# Autodesk Inventor assembly: YZ-Axis Connection
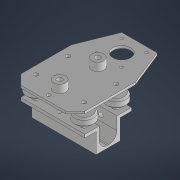
[picture p0: Inventor's stored thumbnail of the model, 180x180]
Saved by Autodesk Inventor 2022 (Build 260153000, 153)
## iProperties
Created: 2023-06-15
Part Number: YZ-Axis Connection
Document SubType Name: Assembly
Designer: Ryan Mitcham
Author: Ryan Mitcham
## Documents named in this file (5)
- C:\Users\Gaming\OneDrive\Documents\Inventor\XYZ-Gantry\YZ-Axis Connection\YZ-Axis Connection.iam
- C:\Users\Gaming\OneDrive\Documents\Inventor\XYZ-Gantry\YZ-Axis Connection\Back Plate.ipt
- C:\Users\Gaming\OneDrive\Documents\Inventor\XYZ-Gantry\YZ-Axis Connection\Back Plate Spacer.ipt
- C:\Users\Gaming\OneDrive\Documents\Inventor\XYZ-Gantry\YZ-Axis Connection\Wheel Mount.ipt
- C:\Users\Gaming\OneDrive\Documents\Inventor\XYZ-Gantry\Standard Parts\20x20 Extrusion Compatible Wheel - Dual Spacers.ipt
## Components (8 placed, 4 different names)
1. Back Plate:1 — Mate:1, Mate:2, Mate:3, Mate:4, Mate:5, Mate:6, Mate:7, Mate:8, Mate:9, Mate:10, Mate:11, Mate:12
2. Back Plate Spacer:1 — Mate:1, Mate:4
3. Back Plate Spacer:2 — Mate:2, Mate:3
4. Wheel Mount:1 — Mate:13, Mate:14, Mate:15, Mate:16, Mate:17, Mate:18, Mate:19
5. 20x20 Extrusion Compatible Wheel - Dual Spacers:1 — Mate:5, Mate:8, Mate:16
6. 20x20 Extrusion Compatible Wheel - Dual Spacers:2 — Mate:6, Mate:7, Mate:13, Mate:14
7. 20x20 Extrusion Compatible Wheel - Dual Spacers:3 — Mate:9, Mate:12, Mate:15
8. 20x20 Extrusion Compatible Wheel - Dual Spacers:4 — Mate:10, Mate:11
## Relationships (19: Mate 19)
- Mate:1: Back Plate:1 ↔ Back Plate Spacer:1
- Mate:2: Back Plate:1 ↔ Back Plate Spacer:2
- Mate:3: Back Plate:1 ↔ Back Plate Spacer:2
- Mate:4: Back Plate:1 ↔ Back Plate Spacer:1
- Mate:5: Back Plate:1 ↔ 20x20 Extrusion Compatible Wheel - Dual Spacers:1
- Mate:6: Back Plate:1 ↔ 20x20 Extrusion Compatible Wheel - Dual Spacers:2
- Mate:7: Back Plate:1 ↔ 20x20 Extrusion Compatible Wheel - Dual Spacers:2
- Mate:8: Back Plate:1 ↔ 20x20 Extrusion Compatible Wheel - Dual Spacers:1
- Mate:9: Back Plate:1 ↔ 20x20 Extrusion Compatible Wheel - Dual Spacers:3
- Mate:10: Back Plate:1 ↔ 20x20 Extrusion Compatible Wheel - Dual Spacers:4
- Mate:11: Back Plate:1 ↔ 20x20 Extrusion Compatible Wheel - Dual Spacers:4
- Mate:12: Back Plate:1 ↔ 20x20 Extrusion Compatible Wheel - Dual Spacers:3
- Mate:13: Wheel Mount:1 ↔ 20x20 Extrusion Compatible Wheel - Dual Spacers:2
- Mate:14: Wheel Mount:1 ↔ 20x20 Extrusion Compatible Wheel - Dual Spacers:2
- Mate:15: Wheel Mount:1 ↔ 20x20 Extrusion Compatible Wheel - Dual Spacers:3
- Mate:16: Wheel Mount:1 ↔ 20x20 Extrusion Compatible Wheel - Dual Spacers:1
- Mate:17: Wheel Mount:1
- Mate:18: Wheel Mount:1
- Mate:19: Wheel Mount:1
